# Autodesk Inventor assembly: stepperToAxleConnectorAssembly
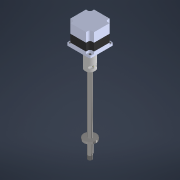
[picture p0: Inventor's stored thumbnail of the model, 180x180]
Saved by Autodesk Inventor 2021.4 (Build 254397000, 397)
## iProperties
Created: 2022-03-02
Part Number: stepperToAxleConnectorAssembly
Document SubType Name: Assembly
Designer: jo_ki
Author: jo_ki
## Documents named in this file (6)
- D:\Repos\SmartSoccerTableCAD\Assemblies\stepperToAxleConnectorAssembly.iam
- D:\Repos\SmartSoccerTableCAD\Parts\ballInletWheelAxle.ipt
- D:\Repos\SmartSoccerTableCAD\Parts\Dimensions\Mastersketch.ipt
- D:\Repos\SmartSoccerTableCAD\Import\stepper_am23hs0420-01\stepper_am23hs0420-01.iam
- D:\Repos\SmartSoccerTableCAD\Parts\stepperToAxleConnector_1.ipt
- D:\Repos\SmartSoccerTableCAD\Parts\stepperToAxleConnector_2.ipt
## Components (4 placed, 4 different names)
1. ballInletWheelAxle:1 — Mate:1, Mate:2, Mate:3, Angle:1, Mate:4, Mate:5
2. stepper_am23hs0420-01:1 [sub-assembly] — Mate:3, Angle:1, Angle:2, Mate:4
3. stepperToAxleConnector_1:1 — Mate:5, Mate:6
4. stepperToAxleConnector_2:1
## Relationships (8: Mate 6, Angle 2)
- Mate:1: ballInletWheelAxle:1
- Mate:2: ballInletWheelAxle:1
- Mate:3: ballInletWheelAxle:1 ↔ stepper_am23hs0420-01:1
- Angle:1 (0 deg): ballInletWheelAxle:1 ↔ stepper_am23hs0420-01:1
- Angle:2 (0 deg): stepper_am23hs0420-01:1
- Mate:4 (5 mm): ballInletWheelAxle:1 ↔ stepper_am23hs0420-01:1
- Mate:5: ballInletWheelAxle:1 ↔ stepperToAxleConnector_1:1
- Mate:6: stepperToAxleConnector_1:1
## Named parameters: profile_width = 40 mm, feet_widthCenter = 720 mm, feet_lengthCenter = 1500 mm, feet_length = 746 mm, profile_height = 160 mm, groundPlate_width = 702 mm, groundPlate_length = 1482 mm, handle_distance = 150 mm, handle_amount = 8, handle_offsetTop = 45 mm, handleAxle_diameter = 16 mm, handleHole_diameter = 36 mm, profileTall_innerHeightOffset = 33 mm, profileTallWall_thickness = 3 mm, groundPlate_thickness = 8 mm, ball_size = 33 mm, ball_rollTolerance = 1 mm, glass_thickness = 6 mm, glass_length = 1200 mm, ballInletHole_groundPlateOffsetBottom = 24 mm, ballInletWheel_margin = 10 mm, ballInletWheel_thickness = 31 mm, ballInletWheelBucket_amount = 6, ballInletWheelSlope_angle = 10 deg, goal_width = 224 mm, goal_height = 96 mm, goal_depth = 89 mm, goalCollector_depth = 68 mm, ballRollbackRail_angle = 5 deg, handleAxle_length = 1100 mm, ballInletWheelDriveShaftAxle_diameter = 10 mm, ballInletWheel_diameter = 238.29764 mm, ballInletWheel_offsetTop = 174.68268 mm, ballInletWheel_tolerance = 1 mm, ballInletHole_bottomOffset = 71.5 mm, playAreaWall_height = 130 mm, goalPanel_thickness = 4 mm, goalArea_width = 130 mm, goalCollector_angle = 45 deg, goalCollectorRollback_angle = 45 deg, goalPlayArea_distance = 228 mm, goalPanelFrontInner_innerWidth = 220 mm, goalPanelBackInner_innerWidth = 672 mm, goalPanelSideOuter_width = 141 mm, goalCollectorPanelSide_angel = 45 deg, goalCollectorRollbackPipe_diameter = 35 mm, pipeConnector_wallThickness = 3 mm, pipe_wallThickness = 2 mm, axleSupport_offset = 14.68268 mm, axleSupport_distance = 200 mm
